# Autodesk Inventor assembly: Side_bearings
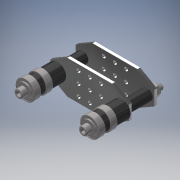
[picture p0: Inventor's stored thumbnail of the model, 180x180]
Saved by Autodesk Inventor 2018 (Build 220112000, 112)
## iProperties
Created: 2018-07-13
Part Number: Side_bearings
Document SubType Name: Assembly
Designer: baoan
Author: baoan
## Documents named in this file (10)
- C:\Users\baoan\Documents\Inventor\Elevator\Side_bearings.iam
- C:\Users\baoan\Documents\Inventor\Elevator\Elevator parts\McMaster-Carr 91251A555_91251A555.ipt
- C:\Users\baoan\Documents\Inventor\Elevator\Elevator parts\McMaster-Carr 90640A129_90640A129.ipt
- C:\Users\baoan\Documents\Inventor\Elevator\Elevator parts\217-2762-001-CUT Rev4_BB2015 1in.ipt
- C:\Users\baoan\Documents\Inventor\Elevator\Side_bearing_flat.ipt
- C:\Users\baoan\Documents\Inventor\Elevator\Elevator parts\McMaster-Carr 92141A029_92141A029.ipt
- C:\Users\baoan\Documents\Inventor\Elevator\Elevator parts\217-3337-001 Rev1.ipt
- C:\Users\baoan\Documents\Inventor\Elevator\Elevator parts\217-2758-001 Rev2.ipt
- C:\Users\baoan\Documents\Inventor\Elevator\Elevator parts\217-3259-001 Rev2.ipt
- C:\Users\baoan\Documents\Inventor\Elevator\Elevator parts\217-3261-001 Rev2.ipt
## Components (20 placed, 9 different names)
1. Side_bearing_flat:1 — Mate:1, Mate:19, Mate:26, Mate:41, Mate:42, Mate:43
2. Side_bearing_flat:2 — Mate:17, Mate:18, Mate:21, Mate:44
3. McMaster-Carr 91251A555_91251A555:3 — Mate:1, Mate:2, Mate:3, Mate:4, Mate:5, Mate:10, Mate:12, Mate:16, Mate:18, Mate:20, Mate:24
4. McMaster-Carr 92141A029_92141A029:1 — Mate:2, Mate:5, Mate:6
5. 217-3337-001 Rev1:1 — Mate:3, Mate:6, Mate:8
6. 217-3259-001 Rev2:1 — Mate:4, Mate:8, Mate:23
7. 217-3337-001 Rev1:2 — Mate:10, Mate:13, Mate:23
8. 217-3261-001 Rev2:1 — Mate:12, Mate:13, Mate:25
9. 217-2762-001-CUT Rev4_BB2015 1in:3 — Mate:16, Mate:17, Mate:19
10. McMaster-Carr 90640A129_90640A129:3 — Mate:20, Mate:21
11. 217-2758-001 Rev2:1 — Mate:24, Mate:25, Mate:26
12. McMaster-Carr 91251A555_91251A555:4 — Mate:41
13. McMaster-Carr 92141A029_92141A029:2
14. 217-3337-001 Rev1:3
15. 217-3259-001 Rev2:2
16. 217-3337-001 Rev1:4
17. 217-3261-001 Rev2:2
18. 217-2762-001-CUT Rev4_BB2015 1in:4 — Mate:43
19. McMaster-Carr 90640A129_90640A129:4 — Mate:44
20. 217-2758-001 Rev2:2 — Mate:42
## Relationships (38: Mate 38)
- Mate:1: Side_bearing_flat:1 ↔ McMaster-Carr 91251A555_91251A555:3
- Mate:2: McMaster-Carr 91251A555_91251A555:3 ↔ McMaster-Carr 92141A029_92141A029:1
- Mate:3: McMaster-Carr 91251A555_91251A555:3 ↔ 217-3337-001 Rev1:1
- Mate:4: McMaster-Carr 91251A555_91251A555:3 ↔ 217-3259-001 Rev2:1
- Mate:5: McMaster-Carr 91251A555_91251A555:3 ↔ McMaster-Carr 92141A029_92141A029:1
- Mate:6: McMaster-Carr 92141A029_92141A029:1 ↔ 217-3337-001 Rev1:1
- Mate:8: 217-3337-001 Rev1:1 ↔ 217-3259-001 Rev2:1
- Mate:10: McMaster-Carr 91251A555_91251A555:3 ↔ 217-3337-001 Rev1:2
- Mate:12: McMaster-Carr 91251A555_91251A555:3 ↔ 217-3261-001 Rev2:1
- Mate:13: 217-3337-001 Rev1:2 ↔ 217-3261-001 Rev2:1
- Mate:16: McMaster-Carr 91251A555_91251A555:3 ↔ 217-2762-001-CUT Rev4_BB2015 1in:3
- Mate:17: Side_bearing_flat:2 ↔ 217-2762-001-CUT Rev4_BB2015 1in:3
- Mate:18: Side_bearing_flat:2 ↔ McMaster-Carr 91251A555_91251A555:3
- Mate:19: Side_bearing_flat:1 ↔ 217-2762-001-CUT Rev4_BB2015 1in:3
- Mate:20: McMaster-Carr 91251A555_91251A555:3 ↔ McMaster-Carr 90640A129_90640A129:3
- Mate:21: Side_bearing_flat:2 ↔ McMaster-Carr 90640A129_90640A129:3
- Mate:23: 217-3259-001 Rev2:1 ↔ 217-3337-001 Rev1:2
- Mate:24: McMaster-Carr 91251A555_91251A555:3 ↔ 217-2758-001 Rev2:1
- Mate:25: 217-3261-001 Rev2:1 ↔ 217-2758-001 Rev2:1
- Mate:26: Side_bearing_flat:1 ↔ 217-2758-001 Rev2:1
- [Mate]: McMaster-Carr 91251A555_91251A555:4 ↔ McMaster-Carr 92141A029_92141A029:2
- [Mate]: McMaster-Carr 91251A555_91251A555:4 ↔ 217-3337-001 Rev1:3
- [Mate]: McMaster-Carr 91251A555_91251A555:4 ↔ 217-3259-001 Rev2:2
- [Mate]: McMaster-Carr 91251A555_91251A555:4 ↔ McMaster-Carr 92141A029_92141A029:2
- [Mate]: McMaster-Carr 92141A029_92141A029:2 ↔ 217-3337-001 Rev1:3
- [Mate]: 217-3337-001 Rev1:3 ↔ 217-3259-001 Rev2:2
- [Mate]: McMaster-Carr 91251A555_91251A555:4 ↔ 217-3337-001 Rev1:4
- [Mate]: McMaster-Carr 91251A555_91251A555:4 ↔ 217-3261-001 Rev2:2
- [Mate]: 217-3337-001 Rev1:4 ↔ 217-3261-001 Rev2:2
- [Mate]: McMaster-Carr 91251A555_91251A555:4 ↔ 217-2762-001-CUT Rev4_BB2015 1in:4
- [Mate]: McMaster-Carr 91251A555_91251A555:4 ↔ McMaster-Carr 90640A129_90640A129:4
- [Mate]: 217-3259-001 Rev2:2 ↔ 217-3337-001 Rev1:4
- [Mate]: McMaster-Carr 91251A555_91251A555:4 ↔ 217-2758-001 Rev2:2
- [Mate]: 217-3261-001 Rev2:2 ↔ 217-2758-001 Rev2:2
- Mate:41: Side_bearing_flat:1 ↔ McMaster-Carr 91251A555_91251A555:4
- Mate:42: Side_bearing_flat:1 ↔ 217-2758-001 Rev2:2
- Mate:43: Side_bearing_flat:1 ↔ 217-2762-001-CUT Rev4_BB2015 1in:4
- Mate:44: Side_bearing_flat:2 ↔ McMaster-Carr 90640A129_90640A129:4
## Named parameters: d114_d109 = 0 mm, d115_d111 = 0 mm, d116_d112 = 0 mm, d117_d94 = 0 mm, d118_d96 = 0 mm, d119_d98 = 0 mm, d120_d99 = 0 mm, d121_d102 = 0 mm, d122_d106 = 0 mm, d123_d88 = 0 mm, d124_d89 = 0 mm, d125_d90 = 0 mm, d126_d91 = 0 mm, d127_d92 = 0 mm
